# Autodesk Inventor assembly: Rebreather-Endcap-Assy
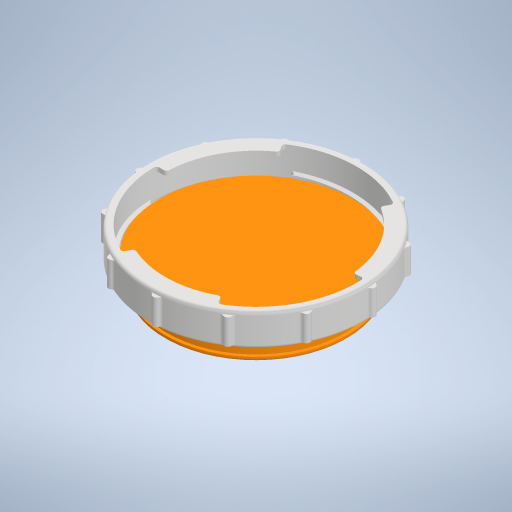
[picture p0: Inventor's stored thumbnail of the model, 512x512]
Saved by Autodesk Inventor 2023 (Build 270158000, 158)
## iProperties
Created: 2022-11-10
Part Number: Rebreather-Endcap-Assy
Document SubType Name: Assembly
Designer: incep
Author: incep
## Documents named in this file (3)
- C:\Projects\rebreather\Rebreather-Endcap-Assy.iam
- C:\Projects\rebreather\Rebreather-Endcap-Insert.ipt
- C:\Projects\rebreather\Rebreather-Endcap-Ring.ipt
## Components (2 placed, 2 different names)
1. Rebreather-Endcap-Insert:1 — Mate:1, Flush:1
2. Rebreather-Endcap-Ring:1 — Mate:2
## Relationships (3: Mate 2, Flush 1)
- Mate:1: Rebreather-Endcap-Insert:1
- Flush:1: Rebreather-Endcap-Insert:1
- Mate:2: Rebreather-Endcap-Ring:1
